# Autodesk Inventor assembly: obudowa - budzik
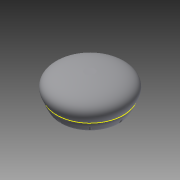
[picture p0: Inventor's stored thumbnail of the model, 180x180]
Saved by Autodesk Inventor 2014 (Build 180170000, 170)
## iProperties
Created: 2018-02-28
Part Number: obudowa - budzik
Document SubType Name: Assembly
Designer: HP820
Author: HP820
## Documents named in this file (3)
- C:\Users\HP820\Dysk Google\Projekt SYSTEM POWIADOMIEN DLA OSOB GLUCHONIEMYCH I NIEDOSLYSZACYCH BY JACEK MARTYNIAK I ŁUKASZ NOWARKIEWICZ\Projekty 3D obudowy\obudowa - budzik\obudowa - budzik.iam
- C:\Users\HP820\Dysk Google\Projekt SYSTEM POWIADOMIEN DLA OSOB GLUCHONIEMYCH I NIEDOSLYSZACYCH BY JACEK MARTYNIAK I ŁUKASZ NOWARKIEWICZ\Projekty 3D obudowy\obudowa - budzik\obudowa - budzik - podstawa.ipt
- C:\Users\HP820\Dysk Google\Projekt SYSTEM POWIADOMIEN DLA OSOB GLUCHONIEMYCH I NIEDOSLYSZACYCH BY JACEK MARTYNIAK I ŁUKASZ NOWARKIEWICZ\Projekty 3D obudowy\obudowa - budzik\obudowa - budzik - gora.ipt
## Components (2 placed, 2 different names)
1. obudowa - budzik - podstawa:1 — Flush:1, Flush:2, Flush:3, Flush:4
2. obudowa - budzik - gora:1 — Flush:1, Flush:2, Flush:3, Flush:4
## Relationships (4: Flush 4)
- Flush:1: obudowa - budzik - podstawa:1 ↔ obudowa - budzik - gora:1
- Flush:2 (45.25 mm): obudowa - budzik - podstawa:1 ↔ obudowa - budzik - gora:1
- Flush:3 (9.5 mm): obudowa - budzik - podstawa:1 ↔ obudowa - budzik - gora:1
- Flush:4: obudowa - budzik - podstawa:1 ↔ obudowa - budzik - gora:1
